# Autodesk Inventor assembly: Gear HS 84 tooth (fixed)
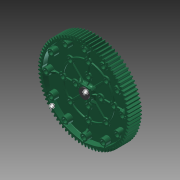
[picture p0: Inventor's stored thumbnail of the model, 180x180]
Saved by Autodesk Inventor 2015 (Build 190159000, 159)
## iProperties
Created: 2014-05-17
Part Number: Gear HS 84 tooth (fixed)
Document SubType Name: Assembly
Designer: Christopher
Author: Christopher
## Documents named in this file (3)
- F:\VEX CAD Library\Motion\Gear HS 84 tooth (fixed).iam
- F:\VEX CAD Library\Motion\Gear HS 84 tooth.ipt
- F:\VEX CAD Library\Motion\Insert HS Metal.ipt
## Components (3 placed, 2 different names)
1. Gear HS 84 tooth:1 — Mate:1, Mate:2, Angle:1, Angle:2, Mate:3, Mate:4
2. Insert HS Metal:1 — Angle:2, Mate:3, Mate:4
3. Insert HS Metal:2 — Mate:1, Mate:2, Angle:1
## Relationships (6: Mate 4, Angle 2)
- Mate:1: Gear HS 84 tooth:1 ↔ Insert HS Metal:2
- Mate:2: Gear HS 84 tooth:1 ↔ Insert HS Metal:2
- Angle:1 (0 deg): Gear HS 84 tooth:1 ↔ Insert HS Metal:2
- Angle:2 (0 deg): Gear HS 84 tooth:1 ↔ Insert HS Metal:1
- Mate:3: Gear HS 84 tooth:1 ↔ Insert HS Metal:1
- Mate:4: Gear HS 84 tooth:1 ↔ Insert HS Metal:1
